# Autodesk Inventor assembly: 000 Ensamblaje 3d_DAA - BASIC
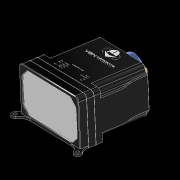
[picture p0: Inventor's stored thumbnail of the model, 180x180]
Saved by Autodesk Inventor 2018 (Build 220112000, 112)
## iProperties
Category: 0
Created: 2024-03-14
Part Number: 000 Ensamblaje 3d_DAA - BASIC
Document SubType Name: Assembly
Designer: cda1
Mass: 217.675 g
Surface Area: 967.459 cm^2
Volume: 79.0664 cm^3
Density: 2.75306 g/cm^3
Manufacturer-1: {"Link": "", "Name": "Embention Sistemas Inteligentes S.A.", "PartNumber": "3d_DAA/BASIC", "partner_id": false}
Manufacturer-2: {"Link": "", "Name": "", "PartNumber": "", "partner_id": false}
Manufacturer-3: {"Link": "", "Name": "", "PartNumber": "", "partner_id": false}
Manufacturer-4: {"Link": "", "Name": "", "PartNumber": "", "partner_id": false}
Manufacturer-5: {"Link": "", "Name": "", "PartNumber": "", "partner_id": false}
Provider-1: {"Link": "", "Name": "Embention Sistemas Inteligentes S.A.", "PartNumber": "3d_DAA/BASIC", "partner_id": 1}
Provider-2: {"Link": "", "Name": "", "PartNumber": "", "partner_id": false}
Provider-3: {"Link": "", "Name": "", "PartNumber": "", "partner_id": false}
Provider-4: {"Link": "", "Name": "", "PartNumber": "", "partner_id": false}
Provider-5: {"Link": "", "Name": "", "PartNumber": "", "partner_id": false}
odoo_id: 15698
odoo_item_code: 3d_DAA
odoo_internal_code: P010345
odoo_pt_internal_code: PT08538
odoo_part_number_code: 3d_DAA/BASIC-101010
odoo_model: product.template
odoo_x2o_application_version: 12.0.4.10
odoo_d2o_version: 12.0.1.4.34
Author: cda1
## Documents named in this file (22)
- C:\Users\cda1\Git\DAA\items\3d_DAA\variants\BASIC\000 Ensamblaje 3d_DAA - BASIC.iam
- C:\Users\cda1\Git\DAA\items\3d_DAA\3d\3d_DAA - M12 Lens Mount.ipt
- C:\Users\cda1\Git\DAA\items\_accessories\Tornilleria\Tornillos\3d_DIN 965H\3d\A2 Black Inox\DIN 965H - M2 x 0,4 x 5 - Black Inox.ipt
- C:\Users\cda1\Git\DAA\items\_accessories\Lentes\3d_EdmundOptics\3d\88-590\88-590.ipt
- C:\Users\cda1\Git\DAA\items\_accessories\Estanqueidad\Juntas toricas\3d_Genérico\3d\Junta tórica 10,5x1.ipt
- C:\Users\cda1\Git\DAA\items\_accessories\Estanqueidad\Juntas toricas\3d_Genérico\3d\Junta torica 2 x 4 x 1 en eje de 3mm.ipt
- C:\Users\cda1\Git\DAA\items\_accessories\Cables y conectores\3d_Lemo\3d\HER.LM.368.XLNP\Comercial\HER.LM.368.XLNP.iam
- C:\Users\cda1\Git\DAA\items\_accessories\Tornilleria\Tornillos\3d_DIN 912\3d\A4 Black Inox\DIN 912 - M2 x 0,4 x 12 - Black INOX.ipt
- C:\Users\cda1\Git\DAA\items\hw_DAA\variants\BASIC\3d\000 Ensamblaje hw_DAA - BASIC - Cubo.iam
- C:\Users\cda1\Git\DAA\items\3d_DAA\3d\3d_DAA - Enclosure Glass.ipt
- C:\Users\cda1\Git\DAA\items\3d_DAA\3d\3d_DAA - Enclosure - FRONT.ipt
- C:\Users\cda1\Git\DAA\items\3d_DAA\3d\3d_DAA - Glass mount.ipt
- C:\Users\cda1\Git\DAA\items\3d_DAA\3d\3d_DAA - Enclosure - REAR.ipt
- C:\Users\cda1\Git\DAA\items\_accessories\Tornilleria\Tornillos\3d_ISO 14581\3d\A4 Black Inox\ISO 14581 - M3 x 0,50 x 18 - Black INOX.ipt
- C:\Users\cda1\Git\DAA\items\_accessories\Thermal pad\3d_Taica\3d\1\Thermal pad 1mm 35x35mm.ipt
- C:\Users\cda1\Git\DAA\items\_accessories\Thermal pad\3d_Taica\3d\3\3mm Thermal Pad 43.5x27mm.ipt
- C:\Users\cda1\Git\DAA\items\_accessories\Thermal pad\3d_Taica\3d\0.5\0.5mm Thermal Pad 43.5x27mm.ipt
- C:\Users\cda1\Git\DAA\items\_accessories\Thermal pad\3d_Taica\3d\1\Thermal pad 1mm 7.5x7.5mm.ipt
- C:\Users\cda1\Git\DAA\items\3d_DAA\3d\3d_DAA - Enclosure - REAR - Phantom.ipt
- C:\Users\cda1\Git\DAA\items\_accessories\Memorias\Micro SD\3d_ATP\3d\ATP-FT128GUD4APEBFI-EMB1.ipt
- C:\Users\cda1\Git\DAA\items\_accessories\Estanqueidad\Juntas toricas\3d_Genérico\3d\Junta tórica 60x1.ipt
- C:\Users\cda1\Git\DAA\items\3d_DAA\3d\3d_DAA - Glass o-ring 60x1.ipt
## Components (43 placed, 21 different names)
1. 88-590:1 — Coincidencia:148, Coincidencia:364, Coincidencia:399
2. Junta torica 2 x 4 x 1 en eje de 3mm:4 — Tangente:11, Coincidencia:396
3. Junta torica 2 x 4 x 1 en eje de 3mm:3 — Tangente:13, Coincidencia:395
4. Junta torica 2 x 4 x 1 en eje de 3mm:2 — Tangente:12, Coincidencia:394
5. Junta torica 2 x 4 x 1 en eje de 3mm:1 — Coincidencia:385, Tangente:10
6. ISO 14581 - M3 x 0,50 x 18 - Black INOX:1 — Coincidencia:392, Nivelación:92
7. ISO 14581 - M3 x 0,50 x 18 - Black INOX:2 — Coincidencia:386, Nivelación:90
8. ISO 14581 - M3 x 0,50 x 18 - Black INOX:4 — Coincidencia:385, Coincidencia:393, Nivelación:90, Nivelación:91, Tangente:14
9. ISO 14581 - M3 x 0,50 x 18 - Black INOX:3 — Coincidencia:389, Nivelación:91, Nivelación:92
10. DIN 965H - M2 x 0,4 x 5 - Black Inox:1 — Nivelación:50, Nivelación:51, Coincidencia:355, Nivelación:78
11. DIN 965H - M2 x 0,4 x 5 - Black Inox:2 — Nivelación:50, Coincidencia:350
12. DIN 965H - M2 x 0,4 x 5 - Black Inox:3 — Nivelación:51, Coincidencia:356
13. DIN 965H - M2 x 0,4 x 5 - Black Inox:4 — Coincidencia:349, Nivelación:87
14. DIN 965H - M2 x 0,4 x 5 - Black Inox:5 — Coincidencia:348, Nivelación:86
15. DIN 912 - M2 x 0,4 x 12 - Black INOX:1 — Coincidencia:354, Coincidencia:361
16. DIN 912 - M2 x 0,4 x 12 - Black INOX:2 — Coincidencia:353, Coincidencia:362
17. DIN 912 - M2 x 0,4 x 12 - Black INOX:3 — Coincidencia:352, Coincidencia:363
18. DIN 912 - M2 x 0,4 x 12 - Black INOX:4 — Coincidencia:351, Coincidencia:360
19. DIN 965H - M2 x 0,4 x 5 - Black Inox:6 — Coincidencia:346, Nivelación:81
20. DIN 965H - M2 x 0,4 x 5 - Black Inox:7 — Coincidencia:347, Nivelación:82
21. DIN 965H - M2 x 0,4 x 5 - Black Inox:8 — Coincidencia:341, Nivelación:83
22. DIN 965H - M2 x 0,4 x 5 - Black Inox:9 — Coincidencia:342, Nivelación:84
23. DIN 965H - M2 x 0,4 x 5 - Black Inox:10 — Coincidencia:343, Nivelación:85
24. DIN 965H - M2 x 0,4 x 5 - Black Inox:11 — Coincidencia:345, Nivelación:80
25. DIN 965H - M2 x 0,4 x 5 - Black Inox:12 — Coincidencia:344, Nivelación:79
26. Junta tórica 10,5x1:1 — Coincidencia:291, Tangente:9
27. Thermal pad 1mm 35x35mm:1 — Coincidencia:403, Nivelación:93, Nivelación:94
28. 3mm Thermal Pad 43.5x27mm:1 — Coincidencia:404, Ángulo:4, Nivelación:95, Nivelación:96, Coincidencia:405, Nivelación:97, Nivelación:98
29. 0.5mm Thermal Pad 43.5x27mm:1 — Coincidencia:405, Nivelación:97, Nivelación:98
30. Thermal pad 1mm 7.5x7.5mm:1 — Coincidencia:408
31. Thermal pad 1mm 7.5x7.5mm:2 — Coincidencia:407, Nivelación:99, Nivelación:100
32. Thermal pad 1mm 7.5x7.5mm:3 — Coincidencia:406, Nivelación:101, Nivelación:102
33. Junta tórica 60x1:1
34. 3d_DAA - Glass o-ring 60x1:1 — Tangente:16
35. 3d_DAA - M12 Lens Mount:1 — Coincidencia:148, Coincidencia:291, Tangente:9, Coincidencia:357, Coincidencia:358, Coincidencia:359
36. 3d_DAA - Glass mount:1 — Coincidencia:400, Ángulo:3, Tangente:17, Coincidencia:401
37. 3d_DAA - Enclosure - FRONT:1 — Coincidencia:398, Coincidencia:399, Tangente:16, Coincidencia:409, Coincidencia:410, Coincidencia:411
38. 3d_DAA - Enclosure - REAR:1 — Coincidencia:383, Ángulo:2, Coincidencia:389, Coincidencia:392, Tangente:10, Tangente:11, Tangente:12, Tangente:13, Coincidencia:386, Coincidencia:393, Coincidencia:394, Coincidencia:395, Coincidencia:396, Tangente:14, Coincidencia:398
39. 3d_DAA - Enclosure - REAR - Phantom:1 — Coincidencia:409, Coincidencia:410, Coincidencia:411
40. 3d_DAA - Enclosure Glass:1 — Coincidencia:400, Ángulo:3, Tangente:17, Coincidencia:401
41. 000 Ensamblaje hw_DAA - BASIC - Cubo:1 [sub-assembly] — Coincidencia:341, Coincidencia:342, Coincidencia:343, Coincidencia:344, Coincidencia:345, Coincidencia:346, Coincidencia:347, Coincidencia:348, Coincidencia:349, Coincidencia:350, Coincidencia:351, Coincidencia:352, Coincidencia:353, Coincidencia:354, Coincidencia:355, Coincidencia:356, Coincidencia:357, Coincidencia:358, Coincidencia:359, Nivelación:78, Nivelación:79, Nivelación:80, Nivelación:81, Nivelación:82, Nivelación:83, Nivelación:84, Nivelación:85, Nivelación:86, Nivelación:87, Coincidencia:360, Coincidencia:361, Coincidencia:362, Coincidencia:363, Coincidencia:364, Coincidencia:365, Coincidencia:366, Coincidencia:367, Coincidencia:373, Ángulo:2, Coincidencia:403, Nivelación:93, Nivelación:94, Coincidencia:404, Ángulo:4, Nivelación:95, Nivelación:96, Coincidencia:406, Coincidencia:407, Coincidencia:408, Nivelación:99, Nivelación:100, Nivelación:101, Nivelación:102
42. HER.LM.368.XLNP:1 [sub-assembly] — Coincidencia:365, Coincidencia:366, Coincidencia:367, Coincidencia:383
43. ATP-FT128GUD4APEBFI-EMB1:1 — Coincidencia:373
## Relationships (92: Mate 55, Flush 26, Tangent 8, Angle 3)
- Nivelación:50 [Flush]: DIN 965H - M2 x 0,4 x 5 - Black Inox:1 ↔ DIN 965H - M2 x 0,4 x 5 - Black Inox:2
- Nivelación:51 [Flush]: DIN 965H - M2 x 0,4 x 5 - Black Inox:1 ↔ DIN 965H - M2 x 0,4 x 5 - Black Inox:3
- Coincidencia:148 [Mate]: 88-590:1 ↔ 3d_DAA - M12 Lens Mount:1
- Coincidencia:291 [Mate]: Junta tórica 10,5x1:1 ↔ 3d_DAA - M12 Lens Mount:1
- Tangente:9: Junta tórica 10,5x1:1 ↔ 3d_DAA - M12 Lens Mount:1
- Coincidencia:341 [Mate]: DIN 965H - M2 x 0,4 x 5 - Black Inox:8 ↔ 000 Ensamblaje hw_DAA - BASIC - Cubo:1
- Coincidencia:342 [Mate]: DIN 965H - M2 x 0,4 x 5 - Black Inox:9 ↔ 000 Ensamblaje hw_DAA - BASIC - Cubo:1
- Coincidencia:343 [Mate]: DIN 965H - M2 x 0,4 x 5 - Black Inox:10 ↔ 000 Ensamblaje hw_DAA - BASIC - Cubo:1
- Coincidencia:344 [Mate]: DIN 965H - M2 x 0,4 x 5 - Black Inox:12 ↔ 000 Ensamblaje hw_DAA - BASIC - Cubo:1
- Coincidencia:345 [Mate]: DIN 965H - M2 x 0,4 x 5 - Black Inox:11 ↔ 000 Ensamblaje hw_DAA - BASIC - Cubo:1
- Coincidencia:346 [Mate]: DIN 965H - M2 x 0,4 x 5 - Black Inox:6 ↔ 000 Ensamblaje hw_DAA - BASIC - Cubo:1
- Coincidencia:347 [Mate]: DIN 965H - M2 x 0,4 x 5 - Black Inox:7 ↔ 000 Ensamblaje hw_DAA - BASIC - Cubo:1
- Coincidencia:348 [Mate]: DIN 965H - M2 x 0,4 x 5 - Black Inox:5 ↔ 000 Ensamblaje hw_DAA - BASIC - Cubo:1
- Coincidencia:349 [Mate]: DIN 965H - M2 x 0,4 x 5 - Black Inox:4 ↔ 000 Ensamblaje hw_DAA - BASIC - Cubo:1
- Coincidencia:350 [Mate]: DIN 965H - M2 x 0,4 x 5 - Black Inox:2 ↔ 000 Ensamblaje hw_DAA - BASIC - Cubo:1
- Coincidencia:351 [Mate]: DIN 912 - M2 x 0,4 x 12 - Black INOX:4 ↔ 000 Ensamblaje hw_DAA - BASIC - Cubo:1
- Coincidencia:352 [Mate]: DIN 912 - M2 x 0,4 x 12 - Black INOX:3 ↔ 000 Ensamblaje hw_DAA - BASIC - Cubo:1
- Coincidencia:353 [Mate]: DIN 912 - M2 x 0,4 x 12 - Black INOX:2 ↔ 000 Ensamblaje hw_DAA - BASIC - Cubo:1
- Coincidencia:354 [Mate]: DIN 912 - M2 x 0,4 x 12 - Black INOX:1 ↔ 000 Ensamblaje hw_DAA - BASIC - Cubo:1
- Coincidencia:355 [Mate]: DIN 965H - M2 x 0,4 x 5 - Black Inox:1 ↔ 000 Ensamblaje hw_DAA - BASIC - Cubo:1
- Coincidencia:356 [Mate]: DIN 965H - M2 x 0,4 x 5 - Black Inox:3 ↔ 000 Ensamblaje hw_DAA - BASIC - Cubo:1
- Coincidencia:357 [Mate]: 3d_DAA - M12 Lens Mount:1 ↔ 000 Ensamblaje hw_DAA - BASIC - Cubo:1
- Coincidencia:358 [Mate]: 3d_DAA - M12 Lens Mount:1 ↔ 000 Ensamblaje hw_DAA - BASIC - Cubo:1
- Coincidencia:359 [Mate]: 3d_DAA - M12 Lens Mount:1 ↔ 000 Ensamblaje hw_DAA - BASIC - Cubo:1
- Nivelación:78 [Flush]: DIN 965H - M2 x 0,4 x 5 - Black Inox:1 ↔ 000 Ensamblaje hw_DAA - BASIC - Cubo:1
- Nivelación:79 [Flush]: DIN 965H - M2 x 0,4 x 5 - Black Inox:12 ↔ 000 Ensamblaje hw_DAA - BASIC - Cubo:1
- Nivelación:80 [Flush]: DIN 965H - M2 x 0,4 x 5 - Black Inox:11 ↔ 000 Ensamblaje hw_DAA - BASIC - Cubo:1
- Nivelación:81 [Flush]: DIN 965H - M2 x 0,4 x 5 - Black Inox:6 ↔ 000 Ensamblaje hw_DAA - BASIC - Cubo:1
- Nivelación:82 [Flush]: DIN 965H - M2 x 0,4 x 5 - Black Inox:7 ↔ 000 Ensamblaje hw_DAA - BASIC - Cubo:1
- Nivelación:83 [Flush]: DIN 965H - M2 x 0,4 x 5 - Black Inox:8 ↔ 000 Ensamblaje hw_DAA - BASIC - Cubo:1
- Nivelación:84 [Flush]: DIN 965H - M2 x 0,4 x 5 - Black Inox:9 ↔ 000 Ensamblaje hw_DAA - BASIC - Cubo:1
- Nivelación:85 [Flush]: DIN 965H - M2 x 0,4 x 5 - Black Inox:10 ↔ 000 Ensamblaje hw_DAA - BASIC - Cubo:1
- Nivelación:86 [Flush]: DIN 965H - M2 x 0,4 x 5 - Black Inox:5 ↔ 000 Ensamblaje hw_DAA - BASIC - Cubo:1
- Nivelación:87 [Flush]: DIN 965H - M2 x 0,4 x 5 - Black Inox:4 ↔ 000 Ensamblaje hw_DAA - BASIC - Cubo:1
- Coincidencia:360 [Mate]: DIN 912 - M2 x 0,4 x 12 - Black INOX:4 ↔ 000 Ensamblaje hw_DAA - BASIC - Cubo:1
- Coincidencia:361 [Mate]: DIN 912 - M2 x 0,4 x 12 - Black INOX:1 ↔ 000 Ensamblaje hw_DAA - BASIC - Cubo:1
- Coincidencia:362 [Mate]: DIN 912 - M2 x 0,4 x 12 - Black INOX:2 ↔ 000 Ensamblaje hw_DAA - BASIC - Cubo:1
- Coincidencia:363 [Mate]: DIN 912 - M2 x 0,4 x 12 - Black INOX:3 ↔ 000 Ensamblaje hw_DAA - BASIC - Cubo:1
- Coincidencia:364 [Mate] (4.8 mm): 88-590:1 ↔ 000 Ensamblaje hw_DAA - BASIC - Cubo:1
- Coincidencia:365 [Mate]: 000 Ensamblaje hw_DAA - BASIC - Cubo:1 ↔ HER.LM.368.XLNP:1
- Coincidencia:366 [Mate]: 000 Ensamblaje hw_DAA - BASIC - Cubo:1 ↔ HER.LM.368.XLNP:1
- Coincidencia:367 [Mate]: 000 Ensamblaje hw_DAA - BASIC - Cubo:1 ↔ HER.LM.368.XLNP:1
- Coincidencia:373 [Mate]: 000 Ensamblaje hw_DAA - BASIC - Cubo:1 ↔ ATP-FT128GUD4APEBFI-EMB1:1
- [Mate]: 3d_DAA - Enclosure - FRONT:1 ↔ 3d_DAA - Enclosure - REAR:1
- [Flush]: 3d_DAA - Enclosure - FRONT:1 ↔ 3d_DAA - Enclosure - REAR:1
- [Mate]: 3d_DAA - Glass mount:1 ↔ 3d_DAA - Enclosure - REAR:1
- [Mate]: 3d_DAA - Glass mount:1 ↔ 3d_DAA - Enclosure - FRONT:1
- Coincidencia:383 [Mate]: 3d_DAA - Enclosure - REAR:1 ↔ HER.LM.368.XLNP:1
- Ángulo:2 [Angle] (0 deg): 3d_DAA - Enclosure - REAR:1 ↔ 000 Ensamblaje hw_DAA - BASIC - Cubo:1
- Coincidencia:385 [Mate]: Junta torica 2 x 4 x 1 en eje de 3mm:1 ↔ ISO 14581 - M3 x 0,50 x 18 - Black INOX:4
- Coincidencia:386 [Mate]: ISO 14581 - M3 x 0,50 x 18 - Black INOX:2 ↔ 3d_DAA - Enclosure - REAR:1
- Coincidencia:389 [Mate]: ISO 14581 - M3 x 0,50 x 18 - Black INOX:3 ↔ 3d_DAA - Enclosure - REAR:1
- Coincidencia:392 [Mate]: ISO 14581 - M3 x 0,50 x 18 - Black INOX:1 ↔ 3d_DAA - Enclosure - REAR:1
- Tangente:10: Junta torica 2 x 4 x 1 en eje de 3mm:1 ↔ 3d_DAA - Enclosure - REAR:1
- Tangente:11: Junta torica 2 x 4 x 1 en eje de 3mm:4 ↔ 3d_DAA - Enclosure - REAR:1
- Tangente:12: Junta torica 2 x 4 x 1 en eje de 3mm:2 ↔ 3d_DAA - Enclosure - REAR:1
- Tangente:13: Junta torica 2 x 4 x 1 en eje de 3mm:3 ↔ 3d_DAA - Enclosure - REAR:1
- Coincidencia:393 [Mate]: ISO 14581 - M3 x 0,50 x 18 - Black INOX:4 ↔ 3d_DAA - Enclosure - REAR:1
- Nivelación:90 [Flush]: ISO 14581 - M3 x 0,50 x 18 - Black INOX:2 ↔ ISO 14581 - M3 x 0,50 x 18 - Black INOX:4
- Nivelación:91 [Flush]: ISO 14581 - M3 x 0,50 x 18 - Black INOX:4 ↔ ISO 14581 - M3 x 0,50 x 18 - Black INOX:3
- Nivelación:92 [Flush]: ISO 14581 - M3 x 0,50 x 18 - Black INOX:1 ↔ ISO 14581 - M3 x 0,50 x 18 - Black INOX:3
- Coincidencia:394 [Mate]: Junta torica 2 x 4 x 1 en eje de 3mm:2 ↔ 3d_DAA - Enclosure - REAR:1
- Coincidencia:395 [Mate]: Junta torica 2 x 4 x 1 en eje de 3mm:3 ↔ 3d_DAA - Enclosure - REAR:1
- Coincidencia:396 [Mate]: Junta torica 2 x 4 x 1 en eje de 3mm:4 ↔ 3d_DAA - Enclosure - REAR:1
- Tangente:14: ISO 14581 - M3 x 0,50 x 18 - Black INOX:4 ↔ 3d_DAA - Enclosure - REAR:1
- Coincidencia:398 [Mate]: 3d_DAA - Enclosure - FRONT:1 ↔ 3d_DAA - Enclosure - REAR:1
- Coincidencia:399 [Mate]: 88-590:1 ↔ 3d_DAA - Enclosure - FRONT:1
- Tangente:16: 3d_DAA - Glass o-ring 60x1:1 ↔ 3d_DAA - Enclosure - FRONT:1
- Coincidencia:400 [Mate]: 3d_DAA - Glass mount:1 ↔ 3d_DAA - Enclosure Glass:1
- Ángulo:3 [Angle] (0 deg): 3d_DAA - Glass mount:1 ↔ 3d_DAA - Enclosure Glass:1
- Tangente:17 (0.106 mm): 3d_DAA - Glass mount:1 ↔ 3d_DAA - Enclosure Glass:1
- Coincidencia:401 [Mate]: 3d_DAA - Glass mount:1 ↔ 3d_DAA - Enclosure Glass:1
- Coincidencia:403 [Mate]: Thermal pad 1mm 35x35mm:1 ↔ 000 Ensamblaje hw_DAA - BASIC - Cubo:1
- Nivelación:93 [Flush]: Thermal pad 1mm 35x35mm:1 ↔ 000 Ensamblaje hw_DAA - BASIC - Cubo:1
- Nivelación:94 [Flush]: Thermal pad 1mm 35x35mm:1 ↔ 000 Ensamblaje hw_DAA - BASIC - Cubo:1
- Coincidencia:404 [Mate]: 3mm Thermal Pad 43.5x27mm:1 ↔ 000 Ensamblaje hw_DAA - BASIC - Cubo:1
- Ángulo:4 [Angle] (0 deg): 3mm Thermal Pad 43.5x27mm:1 ↔ 000 Ensamblaje hw_DAA - BASIC - Cubo:1
- Nivelación:95 [Flush]: 3mm Thermal Pad 43.5x27mm:1 ↔ 000 Ensamblaje hw_DAA - BASIC - Cubo:1
- Nivelación:96 [Flush]: 3mm Thermal Pad 43.5x27mm:1 ↔ 000 Ensamblaje hw_DAA - BASIC - Cubo:1
- Coincidencia:405 [Mate]: 3mm Thermal Pad 43.5x27mm:1 ↔ 0.5mm Thermal Pad 43.5x27mm:1
- Nivelación:97 [Flush]: 3mm Thermal Pad 43.5x27mm:1 ↔ 0.5mm Thermal Pad 43.5x27mm:1
- Nivelación:98 [Flush]: 3mm Thermal Pad 43.5x27mm:1 ↔ 0.5mm Thermal Pad 43.5x27mm:1
- Coincidencia:406 [Mate]: Thermal pad 1mm 7.5x7.5mm:3 ↔ 000 Ensamblaje hw_DAA - BASIC - Cubo:1
- Coincidencia:407 [Mate]: Thermal pad 1mm 7.5x7.5mm:2 ↔ 000 Ensamblaje hw_DAA - BASIC - Cubo:1
- Coincidencia:408 [Mate]: Thermal pad 1mm 7.5x7.5mm:1 ↔ 000 Ensamblaje hw_DAA - BASIC - Cubo:1
- Nivelación:99 [Flush]: Thermal pad 1mm 7.5x7.5mm:2 ↔ 000 Ensamblaje hw_DAA - BASIC - Cubo:1
- Nivelación:100 [Flush]: Thermal pad 1mm 7.5x7.5mm:2 ↔ 000 Ensamblaje hw_DAA - BASIC - Cubo:1
- Nivelación:101 [Flush]: Thermal pad 1mm 7.5x7.5mm:3 ↔ 000 Ensamblaje hw_DAA - BASIC - Cubo:1
- Nivelación:102 [Flush]: Thermal pad 1mm 7.5x7.5mm:3 ↔ 000 Ensamblaje hw_DAA - BASIC - Cubo:1
- Coincidencia:409 [Mate]: 3d_DAA - Enclosure - FRONT:1 ↔ 3d_DAA - Enclosure - REAR - Phantom:1
- Coincidencia:410 [Mate]: 3d_DAA - Enclosure - FRONT:1 ↔ 3d_DAA - Enclosure - REAR - Phantom:1
- Coincidencia:411 [Mate]: 3d_DAA - Enclosure - FRONT:1 ↔ 3d_DAA - Enclosure - REAR - Phantom:1
